# Autodesk Inventor assembly: CornerConnectAssyLeft
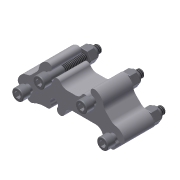
[picture p0: Inventor's stored thumbnail of the model, 180x180]
Saved by Autodesk Inventor 2013 (Build 170138000, 138)
## iProperties
Created: 2012-01-09
Part Number: CornerConnectAssyLeft
Document SubType Name: Assembly
Designer: Nemo
Author: Nemo
## Documents named in this file (4)
- \\lmss\STUDENTS\Robotics\CAD Files\COTS Parts\Kit Frame - AndyMark\Components\CornerConnectAssyLeft.iam
- \\lmss\STUDENTS\Robotics\CAD Files\COTS Parts\Fasteners\14-20 locknut.ipt
- \\lmss\STUDENTS\Robotics\CAD Files\COTS Parts\Kit Frame - AndyMark\Components\Chassis Corner Connect.ipt
- \\lmss\STUDENTS\Robotics\CAD Files\COTS Parts\Fasteners\14-20 SHCS x1750.ipt
## Components (9 placed, 3 different names)
1. Chassis Corner Connect:1 — Insert:15, Insert:16, Insert:17, Insert:18, Insert:19, Insert:20, Insert:21, Insert:22
2. 14-20 locknut:5 — Insert:15
3. 14-20 locknut:6 — Insert:16
4. 14-20 locknut:7 — Insert:18
5. 14-20 locknut:8 — Insert:17
6. Hexagon Socket Head Cap Screw - Inch 1/4 - 20 UNC - 1 3/4:1 — Insert:19
7. Hexagon Socket Head Cap Screw - Inch 1/4 - 20 UNC - 1 3/4:2 — Insert:22
8. Hexagon Socket Head Cap Screw - Inch 1/4 - 20 UNC - 1 3/4:3 — Insert:21
9. Hexagon Socket Head Cap Screw - Inch 1/4 - 20 UNC - 1 3/4:4 — Insert:20
## Relationships (8: Insert 8)
- Insert:15 (3.302 mm): Chassis Corner Connect:1 ↔ 14-20 locknut:5
- Insert:16 (3.302 mm): Chassis Corner Connect:1 ↔ 14-20 locknut:6
- Insert:17 (3.302 mm): Chassis Corner Connect:1 ↔ 14-20 locknut:8
- Insert:18 (3.302 mm): Chassis Corner Connect:1 ↔ 14-20 locknut:7
- Insert:19 (3.175 mm): Chassis Corner Connect:1 ↔ Hexagon Socket Head Cap Screw - Inch 1/4 - 20 UNC - 1 3/4:1
- Insert:20 (3.175 mm): Chassis Corner Connect:1 ↔ Hexagon Socket Head Cap Screw - Inch 1/4 - 20 UNC - 1 3/4:4
- Insert:21 (3.175 mm): Chassis Corner Connect:1 ↔ Hexagon Socket Head Cap Screw - Inch 1/4 - 20 UNC - 1 3/4:3
- Insert:22 (3.175 mm): Chassis Corner Connect:1 ↔ Hexagon Socket Head Cap Screw - Inch 1/4 - 20 UNC - 1 3/4:2
